# Autodesk Inventor assembly: Cup_Dispenser_Alternative
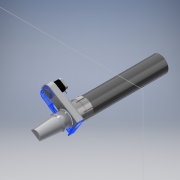
[picture p0: Inventor's stored thumbnail of the model, 180x180]
Saved by Autodesk Inventor 2016 (Build 200138000, 138)
## iProperties
Created: 2015-07-03
Part Number: Cup_Dispenser_Alternative
Document SubType Name: Assembly
Designer: bastli
Author: bastli
## Documents named in this file (8)
- C:\Users\marku\Desktop\Conception\Prototype Construction\Cup_Dispenser_Alternative.iam
- C:\Users\marku\Desktop\Conception\Prototype Construction\Cup_Dispenser_Pipe.ipt
- C:\Users\marku\Desktop\Conception\Prototype Construction\Cup_Dispenser_Cup.ipt
- C:\Users\marku\Desktop\Conception\Prototype Construction\Cup_Dispenser_Pipe_Fixture.ipt
- C:\Users\marku\Documents\Cup_Dispenser_Hull.ipt
- C:\Users\marku\Desktop\Conception\Prototype Construction\Cup_Dispenser_Slider.ipt
- C:\Users\marku\Desktop\Conception\Prototype Construction\M1173041- NEMA 17.ipt
- C:\Users\marku\Documents\Cup_Dispenser_Transmission.ipt
## Components (8 placed, 7 different names)
1. Cup_Dispenser_Pipe:1 — Cylindrical:1, Rigid:1
2. Cup_Dispenser_Cup:1 — Cylindrical:1, Cylindrical:2
3. Cup_Dispenser_Pipe_Fixture:1 — Rigid:1, Rigid:2
4. Cup_Dispenser_Hull:1 — Rigid:2, Rigid:3, Rigid:4
5. Cup_Dispenser_Slider:1 — Rigid:3, Flush:1, Flush:2
6. M1173041- NEMA 17:1 — Rigid:4
7. Cup_Dispenser_Transmission:1 — Flush:1, Flush:2
8. Cup_Dispenser_Cup:2 — Cylindrical:2
## Relationships (8: WeldJoint 4, CylindricalJoint 2, Flush 2)
- Cylindrical:1: Cup_Dispenser_Pipe:1 ↔ Cup_Dispenser_Cup:1
- Rigid:1 [WeldJoint]: Cup_Dispenser_Pipe:1 ↔ Cup_Dispenser_Pipe_Fixture:1
- Rigid:2 [WeldJoint]: Cup_Dispenser_Pipe_Fixture:1 ↔ Cup_Dispenser_Hull:1
- Rigid:3 [WeldJoint]: Cup_Dispenser_Hull:1 ↔ Cup_Dispenser_Slider:1
- Rigid:4 [WeldJoint]: Cup_Dispenser_Hull:1 ↔ M1173041- NEMA 17:1
- Flush:1: Cup_Dispenser_Slider:1 ↔ Cup_Dispenser_Transmission:1
- Flush:2: Cup_Dispenser_Slider:1 ↔ Cup_Dispenser_Transmission:1
- Cylindrical:2: Cup_Dispenser_Cup:1 ↔ Cup_Dispenser_Cup:2
